# Autodesk Inventor assembly: 000 ASY GBK Gubkinskiy
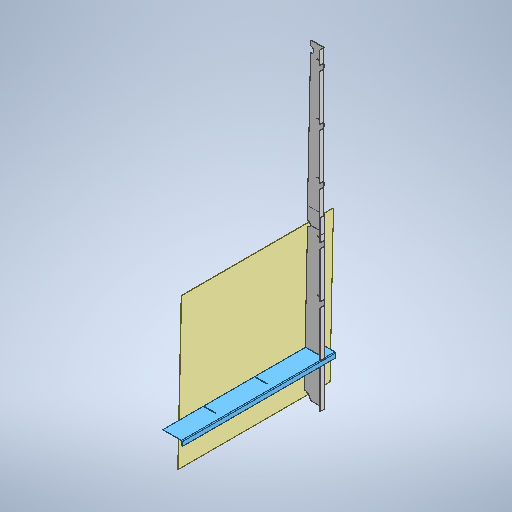
[picture p0: Inventor's stored thumbnail of the model, 512x512]
Saved by Autodesk Inventor 2026.2 (Build 302298000, 298)
## iProperties
Created: 2026-04-17
Part Number: 000 ASY GBK Gubkinskiy
Document SubType Name: Assembly
Designer: admin
Author: admin
## Documents named in this file (9)
- C:\Users\admin\Documents\Inventor\GBK-Gubkinskiy\000 ASY GBK Gubkinskiy.iam
- C:\Users\admin\Documents\Inventor\GBK-Gubkinskiy\GBK bottom.ipt
- C:\Users\admin\Documents\Inventor\GBK-Gubkinskiy\01 ASY GBK wall shield 1.1.1.iam
- C:\Users\admin\Documents\Inventor\GBK-Gubkinskiy\GBK dummy wall 1.ipt
- C:\Users\admin\Documents\Inventor\GBK-Gubkinskiy\GBK dummy wall 4.ipt
- C:\Users\admin\Documents\Inventor\GBK-Gubkinskiy\GBK overall model.ipt
- C:\Users\admin\Documents\Inventor\GBK-Gubkinskiy\01.3 GBK stringer 1.ipt
- C:\Users\admin\Documents\Inventor\GBK-Gubkinskiy\01.2 GBK main rib.ipt
- C:\Users\admin\Documents\Inventor\GBK-Gubkinskiy\02.1 GBK main rib.ipt
## Components (9 placed, 8 different names)
1. 01.2 GBK main rib.ipt:1 — Rotational:1
2. 01.3 GBK stringer 1.ipt:1
3. GBK bottom.ipt:1 — Mate:10, Mate:11, Mate:12, Mate:13, Mate:14, Rigid:1
4. 01 ASY GBK wall shield 1.1.1.iam:1 [sub-assembly]
5. GBK dummy wall 1.ipt:1 — Mate:10
6. GBK dummy wall 1.ipt:2 — Mate:11, Mate:12
7. GBK dummy wall 4.ipt:1 — Mate:13, Mate:14
8. GBK overall model:1 — Rigid:1
9. 02.1 GBK main rib:1 — Rotational:1
## Relationships (13: Mate 8, Flush 2, WeldJoint 2, RevoluteJoint 1)
- [Flush]: GBK bottom.ipt:1 ↔ 01 ASY GBK wall shield 1.1.1.iam:1
- [Mate]: 01.2 GBK main rib.ipt:1 ↔ GBK bottom.ipt:1
- Mate:10: GBK bottom.ipt:1 ↔ GBK dummy wall 1.ipt:1
- Mate:11: GBK bottom.ipt:1 ↔ GBK dummy wall 1.ipt:2
- Mate:12: GBK bottom.ipt:1 ↔ GBK dummy wall 1.ipt:2
- Mate:13: GBK bottom.ipt:1 ↔ GBK dummy wall 4.ipt:1
- Mate:14: GBK bottom.ipt:1 ↔ GBK dummy wall 4.ipt:1
- Rigid:1 [WeldJoint]: GBK bottom.ipt:1 ↔ GBK overall model:1
- [Mate]: 01.2 GBK main rib.ipt:1 ↔ 01 ASY GBK wall shield 1.1.1.iam:1
- [Flush] (250 mm): 01.2 GBK main rib.ipt:1 ↔ 01 ASY GBK wall shield 1.1.1.iam:1
- [Mate]: 01.2 GBK main rib.ipt:1 ↔ 01 ASY GBK wall shield 1.1.1.iam:1
- [WeldJoint] (4 mm): 01.2 GBK main rib.ipt:1 ↔ 01.3 GBK stringer 1.ipt:1
- Rotational:1 [RevoluteJoint]: 01.2 GBK main rib.ipt:1 ↔ 02.1 GBK main rib:1
